# Autodesk Inventor assembly: Tutorial_001_Assembled
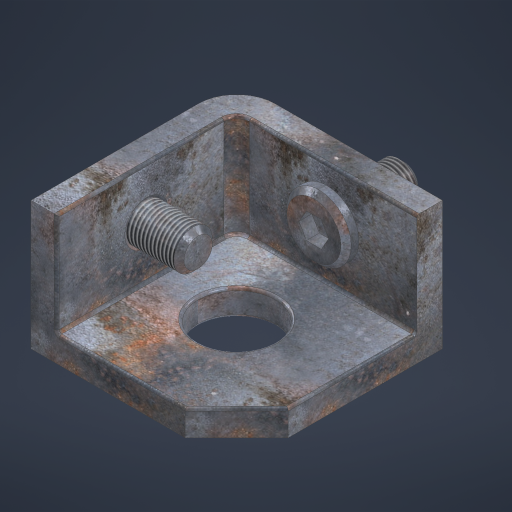
[picture p0: Inventor's stored thumbnail of the model, 512x512]
Saved by Autodesk Inventor 2024.4 (Build 284460000, 460)
## iProperties
Created: 2026-06-08
Part Number: Tutorial_001_Assembled
Document SubType Name: Assembly
Designer: hs4ho
Author: hs4ho
## Documents named in this file (3)
- C:\Users\hs4ho\OneDrive\Documents\GitHub\2026-2027-DesignTraining\DeanS\Tutorial\Tutorial_001_Assembled.iam
- C:\Users\hs4ho\OneDrive\Documents\GitHub\2026-2027-DesignTraining\DeanS\Tutorial\Tutorial_001_Bracket.ipt
- C:\Users\hs4ho\OneDrive\Documents\GitHub\2026-2027-DesignTraining\DeanS\Tutorial\Tutorial_001_Bolt.ipt
## Components (3 placed, 2 different names)
1. Tutorial_001_Bracket:1 — Mate:1, Mate:2, Angle:1, Mate:3, Mate:4, Angle:2
2. Tutorial_001_Bolt:1 — Mate:1, Mate:2, Angle:1
3. Tutorial_001_Bolt:2 — Mate:3, Mate:4, Angle:2
## Relationships (6: Mate 4, Angle 2)
- Mate:1: Tutorial_001_Bracket:1 ↔ Tutorial_001_Bolt:1
- Mate:2: Tutorial_001_Bracket:1 ↔ Tutorial_001_Bolt:1
- Angle:1 (0 deg): Tutorial_001_Bracket:1 ↔ Tutorial_001_Bolt:1
- Mate:3: Tutorial_001_Bracket:1 ↔ Tutorial_001_Bolt:2
- Mate:4: Tutorial_001_Bracket:1 ↔ Tutorial_001_Bolt:2
- Angle:2 (0 deg): Tutorial_001_Bracket:1 ↔ Tutorial_001_Bolt:2
